# Autodesk Inventor assembly: NixieAssem
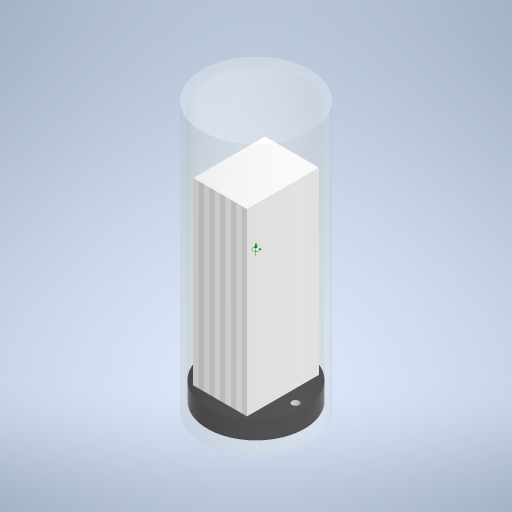
[picture p0: Inventor's stored thumbnail of the model, 512x512]
Saved by Autodesk Inventor 2023 (Build 270158000, 158)
## iProperties
Created: 2022-09-10
Part Number: NixieAssem
Document SubType Name: Assembly
Designer: Desmond
Author: Desmond
## Documents named in this file (5)
- G:\LED Nixie Test\Glass Tube\NixieAssem.iam
- G:\LED Nixie Test\Glass Tube\Acrylic_Seperator.ipt
- G:\LED Nixie Test\Glass Tube\Arcylic_Panel_20mm_1.ipt
- G:\LED Nixie Test\Glass Tube\Arcylic_Panel_20mm_2.ipt
- G:\LED Nixie Test\Glass Tube\Glass_Tube.ipt
## Components (12 placed, 4 different names)
1. Acrylic_Seperator:1 — Mate:1, Mate:2, Flush:1, Mate:3, Mate:4, Flush:2, Flush:3, Mate:5, Mate:6, Mate:7, Mate:8, Flush:4, Mate:9, Flush:5, Mate:10, Mate:11, Mate:12, Flush:6, Mate:13, Mate:14, Flush:7, Mate:15, Flush:8, Mate:16, Mate:17, Flush:9, Mate:18, Mate:19, Flush:10, Mate:20, Mate:21
2. Arcylic_Panel_20mm_1:1 — Mate:1, Mate:2, Flush:1
3. Arcylic_Panel_20mm_1:2 — Flush:3, Mate:5, Mate:6
4. Arcylic_Panel_20mm_1:3 — Mate:3, Mate:4, Flush:2
5. Arcylic_Panel_20mm_1:4 — Mate:9, Flush:5, Mate:10
6. Arcylic_Panel_20mm_1:5 — Mate:7, Mate:8, Flush:4
7. Arcylic_Panel_20mm_2:1 — Mate:13, Mate:14, Flush:7
8. Arcylic_Panel_20mm_2:2 — Mate:15, Flush:8, Mate:16
9. Arcylic_Panel_20mm_2:3 — Mate:17, Flush:9, Mate:18
10. Arcylic_Panel_20mm_2:4 — Mate:19, Flush:10, Mate:20
11. Arcylic_Panel_20mm_2:5 — Mate:11, Mate:12, Flush:6
12. Glass_Tube:1 — Mate:21
## Relationships (31: Mate 21, Flush 10)
- Mate:1: Acrylic_Seperator:1 ↔ Arcylic_Panel_20mm_1:1
- Mate:2: Acrylic_Seperator:1 ↔ Arcylic_Panel_20mm_1:1
- Flush:1: Acrylic_Seperator:1 ↔ Arcylic_Panel_20mm_1:1
- Mate:3: Acrylic_Seperator:1 ↔ Arcylic_Panel_20mm_1:3
- Mate:4: Acrylic_Seperator:1 ↔ Arcylic_Panel_20mm_1:3
- Flush:2: Acrylic_Seperator:1 ↔ Arcylic_Panel_20mm_1:3
- Flush:3: Acrylic_Seperator:1 ↔ Arcylic_Panel_20mm_1:2
- Mate:5: Acrylic_Seperator:1 ↔ Arcylic_Panel_20mm_1:2
- Mate:6: Acrylic_Seperator:1 ↔ Arcylic_Panel_20mm_1:2
- Mate:7: Acrylic_Seperator:1 ↔ Arcylic_Panel_20mm_1:5
- Mate:8: Acrylic_Seperator:1 ↔ Arcylic_Panel_20mm_1:5
- Flush:4: Acrylic_Seperator:1 ↔ Arcylic_Panel_20mm_1:5
- Mate:9: Acrylic_Seperator:1 ↔ Arcylic_Panel_20mm_1:4
- Flush:5: Acrylic_Seperator:1 ↔ Arcylic_Panel_20mm_1:4
- Mate:10: Acrylic_Seperator:1 ↔ Arcylic_Panel_20mm_1:4
- Mate:11: Acrylic_Seperator:1 ↔ Arcylic_Panel_20mm_2:5
- Mate:12: Acrylic_Seperator:1 ↔ Arcylic_Panel_20mm_2:5
- Flush:6: Acrylic_Seperator:1 ↔ Arcylic_Panel_20mm_2:5
- Mate:13: Acrylic_Seperator:1 ↔ Arcylic_Panel_20mm_2:1
- Mate:14: Acrylic_Seperator:1 ↔ Arcylic_Panel_20mm_2:1
- Flush:7: Acrylic_Seperator:1 ↔ Arcylic_Panel_20mm_2:1
- Mate:15: Acrylic_Seperator:1 ↔ Arcylic_Panel_20mm_2:2
- Flush:8: Acrylic_Seperator:1 ↔ Arcylic_Panel_20mm_2:2
- Mate:16: Acrylic_Seperator:1 ↔ Arcylic_Panel_20mm_2:2
- Mate:17: Acrylic_Seperator:1 ↔ Arcylic_Panel_20mm_2:3
- Flush:9: Acrylic_Seperator:1 ↔ Arcylic_Panel_20mm_2:3
- Mate:18: Acrylic_Seperator:1 ↔ Arcylic_Panel_20mm_2:3
- Mate:19: Acrylic_Seperator:1 ↔ Arcylic_Panel_20mm_2:4
- Flush:10: Acrylic_Seperator:1 ↔ Arcylic_Panel_20mm_2:4
- Mate:20: Acrylic_Seperator:1 ↔ Arcylic_Panel_20mm_2:4
- Mate:21: Acrylic_Seperator:1 ↔ Glass_Tube:1
